# Autodesk Inventor assembly: arm_test
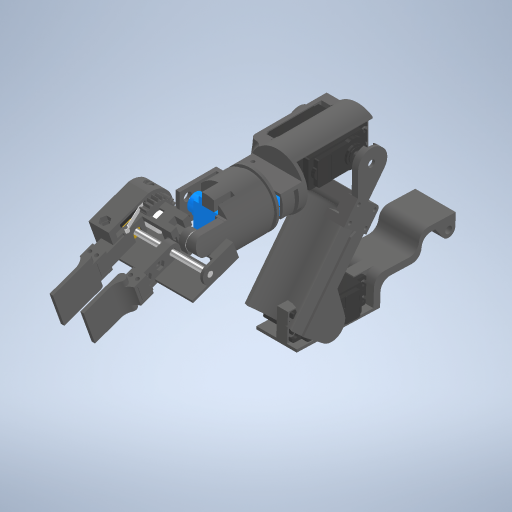
[picture p0: Inventor's stored thumbnail of the model, 512x512]
Saved by Autodesk Inventor 2024.1 (Build 281209000, 209)
## iProperties
Created: 2025-01-27
Part Number: arm_test
Document SubType Name: Assembly
Designer: hibik
Author: hibik
## Documents named in this file (9)
- C:\Users\hibik\Documents\Robomech\RESCUE\ORCA\hard\arm\arm_test.iam
- C:\Users\hibik\Documents\Robomech\RESCUE\ORCA\hard\arm\wrist_wrist.ipt
- C:\Users\hibik\Documents\Robomech\RESCUE\ORCA\hard\std_parts\Miusei_ms18.ipt
- C:\Users\hibik\Documents\Robomech\RESCUE\ORCA\hard\arm\wrist_geard_hone.ipt
- C:\Users\hibik\Documents\Robomech\RESCUE\ORCA\hard\arm\arm_2.ipt
- C:\Users\hibik\Documents\Robomech\RESCUE\ORCA\hard\std_parts\FS5103B.ipt
- C:\Users\hibik\Documents\Robomech\RESCUE\ORCA\hard\arm\arm_1.ipt
- C:\Users\hibik\Documents\Robomech\RESCUE\ORCA\hard\arm\arm_0.ipt
- C:\Users\hibik\Documents\Robomech\RESCUE\ORCA\hard\arm\Assy_hand.iam
## Components (10 placed, 8 different names)
1. wrist_wrist:1 — メイト:1, メイト:2, メイト:3, フラッシュ:2, メイト:4, 挿入:11
2. Miusei_ms18:1 — メイト:1, メイト:2, メイト:3, フラッシュ:1
3. Miusei_ms18:2 — 挿入:1, フラッシュ:1, フラッシュ:2, メイト:4, メイト:5, フラッシュ:3, フラッシュ:4
4. wrist_geard_hone:1 — 挿入:1
5. arm_2:1 — メイト:5, フラッシュ:3, フラッシュ:4, メイト:7, メイト:8, メイト:9
6. FS5103B:1 — メイト:7, メイト:8, 挿入:2, メイト:9
7. arm_1:1 — 挿入:2, 挿入:10
8. arm_0:1 — メイト:10, メイト:11, メイト:12
9. FS5103B:2 — メイト:10, メイト:11, メイト:12, 挿入:10
10. Assy_hand:1 [sub-assembly] — 挿入:11
## Relationships (19: Mate 11, Insert 4, Flush 4)
- メイト:1 [Mate]: wrist_wrist:1 ↔ Miusei_ms18:1
- メイト:2 [Mate]: wrist_wrist:1 ↔ Miusei_ms18:1
- メイト:3 [Mate] (0.1 mm): wrist_wrist:1 ↔ Miusei_ms18:1
- 挿入:1 [Insert]: Miusei_ms18:2 ↔ wrist_geard_hone:1
- フラッシュ:1 [Flush] (5.15 mm): Miusei_ms18:1 ↔ Miusei_ms18:2
- フラッシュ:2 [Flush] (-8 mm): wrist_wrist:1 ↔ Miusei_ms18:2
- メイト:4 [Mate] (2.4 mm): wrist_wrist:1 ↔ Miusei_ms18:2
- メイト:5 [Mate]: Miusei_ms18:2 ↔ arm_2:1
- フラッシュ:3 [Flush]: Miusei_ms18:2 ↔ arm_2:1
- フラッシュ:4 [Flush]: Miusei_ms18:2 ↔ arm_2:1
- メイト:7 [Mate]: arm_2:1 ↔ FS5103B:1
- メイト:8 [Mate]: arm_2:1 ↔ FS5103B:1
- 挿入:2 [Insert]: FS5103B:1 ↔ arm_1:1
- メイト:9 [Mate]: arm_2:1 ↔ FS5103B:1
- メイト:10 [Mate]: arm_0:1 ↔ FS5103B:2
- メイト:11 [Mate]: arm_0:1 ↔ FS5103B:2
- メイト:12 [Mate]: arm_0:1 ↔ FS5103B:2
- 挿入:10 [Insert]: arm_1:1 ↔ FS5103B:2
- 挿入:11 [Insert]: wrist_wrist:1 ↔ Assy_hand:1
